# Autodesk Inventor assembly: Assembly Guitarra 2
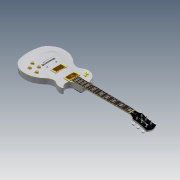
[picture p0: Inventor's stored thumbnail of the model, 180x180]
Saved by Autodesk Inventor 2016 (Build 200138000, 138)
## iProperties
Created: 2018-11-08
Part Number: Assembly Guitarra 2
Document SubType Name: Assembly
Designer: Pedro Mendonça
Author: Pedro Mendonça
## Documents named in this file (27)
- C:\Users\Pedro\Google Drive\Projeto CAD Eng Mecânica\Assembly Guitarra 2.iam
- C:\Users\Pedro\Google Drive\Projeto CAD Eng Mecânica\Corpo.ipt
- C:\Users\Pedro\Google Drive\Projeto CAD Eng Mecânica\Braço.ipt
- C:\Users\Pedro\Google Drive\Projeto CAD Eng Mecânica\Tampo.ipt
- C:\Users\Pedro\Google Drive\Projeto CAD Eng Mecânica\Plug P10 femea.iam
- C:\Users\Pedro\Google Drive\Projeto CAD Eng Mecânica\Arruela POT.ipt
- C:\Users\Pedro\Google Drive\Projeto CAD Eng Mecânica\Potenciometro.ipt
- C:\Users\Pedro\Google Drive\Projeto CAD Eng Mecânica\Porca Potenciometro.ipt
- C:\Users\Pedro\Google Drive\Projeto CAD Eng Mecânica\Knob Assembled.iam
- C:\Users\Pedro\Google Drive\Projeto CAD Eng Mecânica\Base dos parafusos da ponte.ipt
- C:\Users\Pedro\Google Drive\Projeto CAD Eng Mecânica\Segundo Parafuso da Ponte.ipt
- C:\Users\Pedro\Google Drive\Projeto CAD Eng Mecânica\RHYTHM & TREBLE 2.ipt
- C:\Users\Pedro\Google Drive\Projeto CAD Eng Mecânica\Arruela da chave seletora.ipt
- C:\Users\Pedro\Google Drive\Projeto CAD Eng Mecânica\capa de alguma parte da guitarra.ipt
- C:\Users\Pedro\Google Drive\Projeto CAD Eng Mecânica\alguma parte da guitarra.ipt
- C:\Users\Pedro\Google Drive\Projeto CAD Eng Mecânica\Pino da correia.iam
- C:\Users\Pedro\Google Drive\Projeto CAD Eng Mecânica\Tampa inferior.ipt
- C:\Users\Pedro\Google Drive\Projeto CAD Eng Mecânica\Parafuso dos itens externos.ipt
- C:\Users\Pedro\Google Drive\Projeto CAD Eng Mecânica\Tarraxa espelhada.iam
- C:\Users\Pedro\Google Drive\Projeto CAD Eng Mecânica\Tarraxa.iam
- C:\Users\Pedro\Google Drive\Projeto CAD Eng Mecânica\Parafuso Tarraxa.ipt
- C:\Users\Pedro\Google Drive\Projeto CAD Eng Mecânica\Parafuso menor Tarraxa.ipt
- C:\Users\Pedro\Google Drive\Projeto CAD Eng Mecânica\Peça 8 - Montagem.ipt
- C:\Users\Pedro\Google Drive\Projeto CAD Eng Mecânica\Parafuso do Braço.ipt
- C:\Users\Pedro\Google Drive\Projeto CAD Eng Mecânica\Ponte.ipt
- C:\Users\Pedro\Google Drive\Projeto CAD Eng Mecânica\Chave Seletora.ipt
- C:\Users\Pedro\Google Drive\Projeto CAD Eng Mecânica\Porca da Chave Seletora.ipt
## Components (71 placed, 26 different names)
1. Corpo:1 — Cylindrical:2, Cylindrical:3, Rotational:2, Mate:1, Insert:21, Insert:23, Insert:24, Insert:25
2. Braço:1 — Cylindrical:2, Insert:28, Insert:29, Insert:30, Insert:31, Insert:32, Insert:33, Insert:34, Insert:35, Insert:36, Insert:37, Insert:38, Insert:39, Insert:40, Insert:41, Insert:42, Insert:43, Insert:44, Insert:45
3. Tampo:1 — Cylindrical:3, Rigid:1, Rigid:2, Rigid:3, Rigid:4, Insert:13, Insert:14, Insert:15, Insert:16, Insert:19, Insert:52, Insert:53, Insert:54, Insert:55
4. Plug P10 femea:1 [sub-assembly] — Rotational:2
5. Arruela POT:1 — Rigid:1, Insert:2
6. Arruela POT:2 — Rigid:3, Insert:1
7. Arruela POT:3 — Rigid:4, Insert:3
8. Arruela POT:4 — Rigid:2, Insert:4
9. Potenciometro:1 — Insert:1, Insert:6, Insert:9
10. Potenciometro:2 — Insert:3, Insert:5, Insert:10
11. Potenciometro:3 — Insert:4, Insert:8, Insert:12
12. Potenciometro:4 — Insert:2, Insert:7, Insert:11
13. Porca Potenciometro:1 — Insert:6
14. Porca Potenciometro:2 — Insert:7
15. Porca Potenciometro:3 — Insert:5
16. Porca Potenciometro:4 — Insert:8
17. Knob Assembled:1 [sub-assembly] — Insert:11
18. Knob Assembled:2 [sub-assembly] — Insert:12
19. Knob Assembled:3 [sub-assembly] — Insert:10
20. Knob Assembled:4 [sub-assembly] — Insert:9
21. Base dos parafusos da ponte:1 — Insert:13
22. Base dos parafusos da ponte:2 — Insert:14
23. Base dos parafusos da ponte:3 — Insert:16, Insert:17
24. Base dos parafusos da ponte:4 — Insert:15, Insert:18
25. Segundo Parafuso da Ponte:1 — Insert:17, Insert:60
26. Segundo Parafuso da Ponte:2 — Insert:18
27. RHYTHM & TREBLE 2:1 — Insert:19, Insert:20, Insert:61
28. Arruela da chave seletora:1 — Insert:20, Insert:62
29. capa de alguma parte da guitarra:1 — Mate:1, Insert:21, Mate:2, Insert:22
30. alguma parte da guitarra:1 — Mate:2, Insert:22, Insert:56, Insert:57, Insert:58, Insert:59
31. Pino da correia:1 [sub-assembly] — Insert:23
32. Pino da correia:2 [sub-assembly] — Insert:24
33. Tampa inferior:1 — Insert:25, Insert:26, Insert:27
34. Parafuso dos itens externos:1 — Insert:26
35. Parafuso dos itens externos:2
36. Parafuso dos itens externos:3 — Insert:27
37. Tarraxa:1 [sub-assembly] — Insert:36, Insert:37, Insert:50
38. Tarraxa:2 [sub-assembly] — Insert:38, Insert:39, Insert:49
39. Tarraxa:3 [sub-assembly] — Insert:34, Insert:35, Insert:51
40. Tarraxa espelhada:1 [sub-assembly] — Insert:32, Insert:33, Insert:46
41. Tarraxa espelhada:2 [sub-assembly] — Insert:30, Insert:31, Insert:47
42. Tarraxa espelhada:3 [sub-assembly] — Insert:28, Insert:29, Insert:48
43. Parafuso Tarraxa:1 — Insert:42
44. Parafuso Tarraxa:2 — Insert:44
45. Parafuso Tarraxa:3 — Insert:43
46. Parafuso Tarraxa:4 — Insert:45
47. Parafuso Tarraxa:5 — Insert:41
48. Parafuso Tarraxa:6 — Insert:40
49. Parafuso menor Tarraxa:1 — Insert:46
50. Parafuso menor Tarraxa:2 — Insert:47
51. Parafuso menor Tarraxa:3 — Insert:48
52. Parafuso menor Tarraxa:4 — Insert:49
53. Parafuso menor Tarraxa:5 — Insert:50
54. Parafuso menor Tarraxa:6 — Insert:51
55. Peça 8 - Montagem:1 — Insert:54, Insert:55, Insert:67, Insert:68, Insert:69, Insert:70
56. Peça 8 - Montagem:2 — Insert:52, Insert:53, Insert:63, Insert:64, Insert:65, Insert:66
57. Parafuso do Braço:1 — Insert:57
58. Parafuso do Braço:2 — Insert:56
59. Parafuso do Braço:3 — Insert:58
60. Parafuso do Braço:4 — Insert:59
61. Ponte:1 — Insert:60
62. Chave Seletora:2 — Insert:61
63. Porca da Chave Seletora:1 — Insert:62
64. Parafuso dos itens externos:4 — Insert:66
65. Parafuso dos itens externos:5 — Insert:68
66. Parafuso dos itens externos:6 — Insert:69
67. Parafuso dos itens externos:7 — Insert:70
68. Parafuso dos itens externos:8 — Insert:67
69. Parafuso dos itens externos:9 — Insert:65
70. Parafuso dos itens externos:10 — Insert:64
71. Parafuso dos itens externos:11 — Insert:63
## Relationships (79: Insert 70, WeldJoint 4, CylindricalJoint 2, Mate 2, RevoluteJoint 1)
- Cylindrical:2: Corpo:1 ↔ Braço:1
- Cylindrical:3: Corpo:1 ↔ Tampo:1
- Rotational:2 [RevoluteJoint] (-2 mm): Corpo:1 ↔ Plug P10 femea:1
- Rigid:1 [WeldJoint]: Tampo:1 ↔ Arruela POT:1
- Rigid:2 [WeldJoint]: Tampo:1 ↔ Arruela POT:4
- Rigid:3 [WeldJoint]: Tampo:1 ↔ Arruela POT:2
- Rigid:4 [WeldJoint]: Tampo:1 ↔ Arruela POT:3
- Insert:1: Arruela POT:2 ↔ Potenciometro:1
- Insert:2: Arruela POT:1 ↔ Potenciometro:4
- Insert:3: Arruela POT:3 ↔ Potenciometro:2
- Insert:4: Arruela POT:4 ↔ Potenciometro:3
- Insert:5 (-2.5 mm): Potenciometro:2 ↔ Porca Potenciometro:3
- Insert:6 (-3 mm): Potenciometro:1 ↔ Porca Potenciometro:1
- Insert:7 (-3 mm): Potenciometro:4 ↔ Porca Potenciometro:2
- Insert:8 (-3 mm): Potenciometro:3 ↔ Porca Potenciometro:4
- Insert:9: Potenciometro:1 ↔ Knob Assembled:4
- Insert:10 (2 mm): Potenciometro:2 ↔ Knob Assembled:3
- Insert:11: Potenciometro:4 ↔ Knob Assembled:1
- Insert:12 (2 mm): Potenciometro:3 ↔ Knob Assembled:2
- Insert:13 (15.6 mm): Tampo:1 ↔ Base dos parafusos da ponte:1
- Insert:14 (15.6 mm): Tampo:1 ↔ Base dos parafusos da ponte:2
- Insert:15 (15.6 mm): Tampo:1 ↔ Base dos parafusos da ponte:4
- Insert:16 (15.6 mm): Tampo:1 ↔ Base dos parafusos da ponte:3
- Insert:17: Base dos parafusos da ponte:3 ↔ Segundo Parafuso da Ponte:1
- Insert:18: Base dos parafusos da ponte:4 ↔ Segundo Parafuso da Ponte:2
- Insert:19 (3 mm): Tampo:1 ↔ RHYTHM & TREBLE 2:1
- Insert:20: RHYTHM & TREBLE 2:1 ↔ Arruela da chave seletora:1
- Mate:1: Corpo:1 ↔ capa de alguma parte da guitarra:1
- Insert:21: Corpo:1 ↔ capa de alguma parte da guitarra:1
- Mate:2: capa de alguma parte da guitarra:1 ↔ alguma parte da guitarra:1
- Insert:22: capa de alguma parte da guitarra:1 ↔ alguma parte da guitarra:1
- Insert:23 (12 mm): Corpo:1 ↔ Pino da correia:1
- Insert:24 (12 mm): Corpo:1 ↔ Pino da correia:2
- Insert:25: Corpo:1 ↔ Tampa inferior:1
- Insert:26: Tampa inferior:1 ↔ Parafuso dos itens externos:1
- Insert:27: Tampa inferior:1 ↔ Parafuso dos itens externos:3
- Insert:28: Braço:1 ↔ Tarraxa espelhada:3
- Insert:29: Braço:1 ↔ Tarraxa espelhada:3
- Insert:30: Braço:1 ↔ Tarraxa espelhada:2
- Insert:31: Braço:1 ↔ Tarraxa espelhada:2
- Insert:32: Braço:1 ↔ Tarraxa espelhada:1
- Insert:33: Braço:1 ↔ Tarraxa espelhada:1
- Insert:34: Braço:1 ↔ Tarraxa:3
- Insert:35: Braço:1 ↔ Tarraxa:3
- Insert:36: Braço:1 ↔ Tarraxa:1
- Insert:37: Braço:1 ↔ Tarraxa:1
- Insert:38: Braço:1 ↔ Tarraxa:2
- Insert:39: Braço:1 ↔ Tarraxa:2
- Insert:40: Braço:1 ↔ Parafuso Tarraxa:6
- Insert:41: Braço:1 ↔ Parafuso Tarraxa:5
- Insert:42: Braço:1 ↔ Parafuso Tarraxa:1
- Insert:43: Braço:1 ↔ Parafuso Tarraxa:3
- Insert:44: Braço:1 ↔ Parafuso Tarraxa:2
- Insert:45: Braço:1 ↔ Parafuso Tarraxa:4
- Insert:46: Tarraxa espelhada:1 ↔ Parafuso menor Tarraxa:1
- Insert:47: Tarraxa espelhada:2 ↔ Parafuso menor Tarraxa:2
- Insert:48: Tarraxa espelhada:3 ↔ Parafuso menor Tarraxa:3
- Insert:49: Tarraxa:2 ↔ Parafuso menor Tarraxa:4
- Insert:50: Tarraxa:1 ↔ Parafuso menor Tarraxa:5
- Insert:51: Tarraxa:3 ↔ Parafuso menor Tarraxa:6
- Insert:52 (-14 mm): Tampo:1 ↔ Peça 8 - Montagem:2
- Insert:53: Tampo:1 ↔ Peça 8 - Montagem:2
- Insert:54 (-17 mm): Tampo:1 ↔ Peça 8 - Montagem:1
- Insert:55: Tampo:1 ↔ Peça 8 - Montagem:1
- Insert:56: alguma parte da guitarra:1 ↔ Parafuso do Braço:2
- Insert:57: alguma parte da guitarra:1 ↔ Parafuso do Braço:1
- Insert:58: alguma parte da guitarra:1 ↔ Parafuso do Braço:3
- Insert:59: alguma parte da guitarra:1 ↔ Parafuso do Braço:4
- Insert:60: Segundo Parafuso da Ponte:1 ↔ Ponte:1
- Insert:61 (6 mm): RHYTHM & TREBLE 2:1 ↔ Chave Seletora:2
- Insert:62: Arruela da chave seletora:1 ↔ Porca da Chave Seletora:1
- Insert:63: Peça 8 - Montagem:2 ↔ Parafuso dos itens externos:11
- Insert:64: Peça 8 - Montagem:2 ↔ Parafuso dos itens externos:10
- Insert:65: Peça 8 - Montagem:2 ↔ Parafuso dos itens externos:9
- Insert:66: Peça 8 - Montagem:2 ↔ Parafuso dos itens externos:4
- Insert:67: Peça 8 - Montagem:1 ↔ Parafuso dos itens externos:8
- Insert:68: Peça 8 - Montagem:1 ↔ Parafuso dos itens externos:5
- Insert:69: Peça 8 - Montagem:1 ↔ Parafuso dos itens externos:6
- Insert:70: Peça 8 - Montagem:1 ↔ Parafuso dos itens externos:7
